# Autodesk Inventor assembly: SlideAssembly
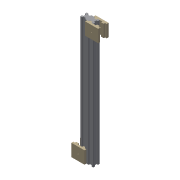
[picture p0: Inventor's stored thumbnail of the model, 180x180]
Saved by Autodesk Inventor 2015 (Build 190159000, 159)
## iProperties
Created: 2015-01-22
Part Number: SlideAssembly
Document SubType Name: Assembly
Designer: rihoobler
Author: rihoobler
## Documents named in this file (3)
- C:\Users\rihoobler\Documents\Inventor\SerenityMk.2\SlideAssembly.iam
- C:\Users\rihoobler\Documents\Inventor\SerenityMk.2\20X40 normal.ipt
- C:\Users\rihoobler\Documents\Inventor\SerenityMk.2\Slider.ipt
## Components (5 placed, 2 different names)
1. 20X40 normal:1 — Flush:1, Mate:1, Mate:2, Mate:3, Mate:4, Mate:5, Flush:3, Mate:6, Mate:7, Flush:4, Mate:8
2. Slider:1 — Flush:1, Mate:1, Mate:2, Flush:2
3. Slider:2 — Flush:2, Mate:3, Mate:4
4. Slider:3 — Mate:7, Flush:4, Mate:8
5. Slider:4 — Mate:5, Flush:3, Mate:6
## Relationships (12: Mate 8, Flush 4)
- Flush:1: 20X40 normal:1 ↔ Slider:1
- Mate:1: 20X40 normal:1 ↔ Slider:1
- Mate:2: 20X40 normal:1 ↔ Slider:1
- Flush:2: Slider:1 ↔ Slider:2
- Mate:3: 20X40 normal:1 ↔ Slider:2
- Mate:4: 20X40 normal:1 ↔ Slider:2
- Mate:5: 20X40 normal:1 ↔ Slider:4
- Flush:3: 20X40 normal:1 ↔ Slider:4
- Mate:6: 20X40 normal:1 ↔ Slider:4
- Mate:7: 20X40 normal:1 ↔ Slider:3
- Flush:4: 20X40 normal:1 ↔ Slider:3
- Mate:8: 20X40 normal:1 ↔ Slider:3
